# Autodesk Inventor assembly: structure_channel
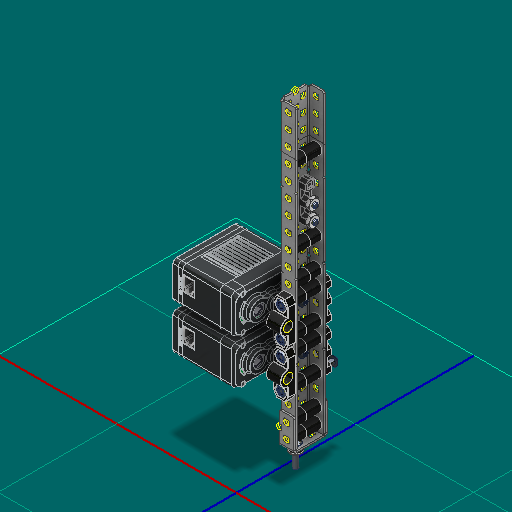
[picture p0: Inventor's stored thumbnail of the model, 512x512]
Saved by Autodesk Inventor 2025 (Build 290162000, 162)
## iProperties
Created: 2024-08-18
Part Number: structure_channel
Document SubType Name: Assembly
Designer: averey
Author: averey
## Documents named in this file (21)
- C:\Users\avere\vex_robotics_high_stakes\hardware\cad\ATLAS\tower\structure\structure_channel.iam
- C:\Users\avere\vex_robotics_high_stakes\hardware\cad\VEX-CAD-Inventor\Structure\C Channel\Aluminum 1x2x1\Alu C 1x2x1x20.ipt
- C:\Users\avere\vex_robotics_high_stakes\hardware\cad\VEX-CAD-Inventor\Structure\C Channel\Aluminum 2x2x2\Alu C 2x2x2x1.ipt
- C:\Users\avere\vex_robotics_high_stakes\hardware\cad\VEX-CAD-Inventor\Motion\Spacers\Spacer Nylon .375 OD\NSpacer .375 OD x .375.ipt
- C:\Users\avere\vex_robotics_high_stakes\hardware\cad\VEX-CAD-Inventor\Motion\Spacers\Spacer Nylon .375 OD.ipt
- C:\Users\avere\vex_robotics_high_stakes\hardware\cad\VEX-CAD-Inventor\Motion\Spacers\Spacer Nylon .375 OD\NSpacer .375 OD x .500.ipt
- C:\Users\avere\vex_robotics_high_stakes\hardware\cad\VEX-CAD-Inventor\Structure\C Channel\Aluminum 1x2x1\Alu C 1x2x1x17.ipt
- C:\Users\avere\vex_robotics_high_stakes\hardware\cad\VEX-CAD-Inventor\Motion\Spacers\Spacer Nylon .375 OD\NSpacer .375 OD x .125.ipt
- C:\Users\avere\vex_robotics_high_stakes\hardware\cad\VEX-CAD-Inventor\Motion\Spacers\Washer Steel\SWasher .375 OD x .015625.ipt
- C:\Users\avere\vex_robotics_high_stakes\hardware\cad\VEX-CAD-Inventor\Motion\Spacers\Washer Steel.ipt
- C:\Users\avere\vex_robotics_high_stakes\hardware\cad\VEX-CAD-Inventor\Motion\Spacers\Washer Steel\SWasher .375 OD x .031250.ipt
- C:\Users\avere\vex_robotics_high_stakes\hardware\cad\VEX-CAD-Inventor\Structure\Hardware\Screw Steel - Star\SScrew Star Smooth .750.ipt
- C:\Users\avere\vex_robotics_high_stakes\hardware\cad\VEX-CAD-Inventor\Structure\Hardware\Screw Steel - Star.ipt
- C:\Users\avere\vex_robotics_high_stakes\hardware\cad\VEX-CAD-Inventor\Electronics\Motors with Screws\SteelM-StarS.iam
- C:\Users\avere\vex_robotics_high_stakes\hardware\cad\VEX-CAD-Inventor\Electronics\Motors with Screws.iam
- C:\Users\avere\vex_robotics_high_stakes\hardware\cad\VEX-CAD-Inventor\Motion\Shaft HS\HS Pillow Bearing Block.ipt
- C:\Users\avere\vex_robotics_high_stakes\hardware\cad\VEX-CAD-Inventor\Motion\Shaft LS\Bearing Flat.ipt
- C:\Users\avere\vex_robotics_high_stakes\hardware\cad\VEX-CAD-Inventor\Structure\Hardware\Screw Steel - Star\SScrew Star Smooth 1.500.ipt
- C:\Users\avere\vex_robotics_high_stakes\hardware\cad\VEX-CAD-Inventor\Structure\Hardware\Nut Thin Nylock.ipt
- C:\Users\avere\vex_robotics_high_stakes\hardware\cad\_quick_assemblies\bearing_flat_w_hardware_offset.iam
- C:\Users\avere\vex_robotics_high_stakes\hardware\cad\VEX-CAD-Inventor\Structure\Hardware\Screw Steel - Star\SScrew Star Smooth 1.750.ipt
## Components (40 placed, 16 different names)
1. Alu C 1x2x1x20:1 — Angle:1, Angle:2, Mate:5, Insert:1, Mate:6, Insert:3, Insert:5, Insert:6, Mate:7
2. Alu C 2x2x2x1:1 — Insert:1, Mate:6, Insert:9, Insert:10
3. NSpacer .375 OD x .375:1 — Insert:2
4. NSpacer .375 OD x .500:2 — Insert:2, Insert:3
5. NSpacer .375 OD x .375:3 — Insert:4
6. NSpacer .375 OD x .500:4 — Insert:4, Insert:5
7. Alu C 1x2x1x17:1 — Insert:6, Mate:7, Insert:11, Mate:8, Insert:12, Mate:9, Insert:15, Mate:12, Insert:16, Mate:13, Insert:18, Insert:20, Insert:22, Insert:24, Insert:25, Mate:14, Insert:26, Mate:15, Insert:35, Mate:16, Insert:37, Insert:39, Insert:41
8. NSpacer .375 OD x .125:5 — Insert:9
9. SWasher .375 OD x .015625:1
10. SWasher .375 OD x .031250:2
11. SScrew Star Smooth .750:1 — Insert:10
12. SteelM-StarS:1 [sub-assembly] — Insert:11, Mate:8
13. SteelM-StarS:2 [sub-assembly] — Insert:12, Mate:9
14. HS Pillow Bearing Block:1 — Insert:15, Mate:12, Insert:31, Insert:32
15. HS Pillow Bearing Block:2 — Insert:16, Mate:13, Insert:33, Insert:34
16. NSpacer .375 OD x .375:6 — Insert:17
17. NSpacer .375 OD x .500:7 — Insert:17, Insert:18
18. NSpacer .375 OD x .375:8
19. NSpacer .375 OD x .500:9 — Insert:20
20. NSpacer .375 OD x .375:10
21. NSpacer .375 OD x .500:11 — Insert:22
22. NSpacer .375 OD x .375:12
23. NSpacer .375 OD x .500:13 — Insert:24
24. Bearing Flat:1 — Insert:25, Mate:14, Insert:29, Insert:42
25. Bearing Flat:2 — Insert:26, Mate:15, Insert:27, Insert:28
26. SScrew Star Smooth 1.500:2 — Insert:27
27. SScrew Star Smooth 1.500:3 — Insert:28
28. SScrew Star Smooth 1.500:5 — Insert:29
29. Nut Thin Nylock:1 — Insert:34
30. Nut Thin Nylock:2 — Insert:32
31. Nut Thin Nylock:3 — Insert:33
32. Nut Thin Nylock:4 — Insert:31
33. bearing_flat_w_hardware_offset:1 [sub-assembly] — Insert:35, Mate:16
34. NSpacer .375 OD x .375:14 — Insert:38
35. NSpacer .375 OD x .500:15 — Insert:38, Insert:39
36. NSpacer .375 OD x .375:16 — Insert:36
37. NSpacer .375 OD x .500:17 — Insert:36, Insert:37
38. NSpacer .375 OD x .375:18
39. NSpacer .375 OD x .500:19 — Insert:41
40. SScrew Star Smooth 1.750:6 — Insert:42
## Relationships (51: Insert 39, Mate 10, Angle 2)
- Angle:1 (0 deg): Alu C 1x2x1x20:1
- Angle:2 (0 deg): Alu C 1x2x1x20:1
- Mate:5 (49.6316 mm): Alu C 1x2x1x20:1
- Insert:1: Alu C 1x2x1x20:1 ↔ Alu C 2x2x2x1:1
- Mate:6: Alu C 1x2x1x20:1 ↔ Alu C 2x2x2x1:1
- Insert:2: NSpacer .375 OD x .375:1 ↔ NSpacer .375 OD x .500:2
- Insert:3: Alu C 1x2x1x20:1 ↔ NSpacer .375 OD x .500:2
- Insert:4: NSpacer .375 OD x .375:3 ↔ NSpacer .375 OD x .500:4
- Insert:5: Alu C 1x2x1x20:1 ↔ NSpacer .375 OD x .500:4
- Insert:6: Alu C 1x2x1x20:1 ↔ Alu C 1x2x1x17:1
- Mate:7: Alu C 1x2x1x20:1 ↔ Alu C 1x2x1x17:1
- [Insert]: SWasher .375 OD x .015625:1 ↔ SWasher .375 OD x .031250:2
- [Insert]: NSpacer .375 OD x .125:5 ↔ SWasher .375 OD x .031250:2
- Insert:9: Alu C 2x2x2x1:1 ↔ NSpacer .375 OD x .125:5
- Insert:10: Alu C 2x2x2x1:1 ↔ SScrew Star Smooth .750:1
- Insert:11: Alu C 1x2x1x17:1 ↔ SteelM-StarS:1
- Mate:8: Alu C 1x2x1x17:1 ↔ SteelM-StarS:1
- Insert:12: Alu C 1x2x1x17:1 ↔ SteelM-StarS:2
- Mate:9: Alu C 1x2x1x17:1 ↔ SteelM-StarS:2
- Insert:15: Alu C 1x2x1x17:1 ↔ HS Pillow Bearing Block:1
- Mate:12: Alu C 1x2x1x17:1 ↔ HS Pillow Bearing Block:1
- Insert:16: Alu C 1x2x1x17:1 ↔ HS Pillow Bearing Block:2
- Mate:13: Alu C 1x2x1x17:1 ↔ HS Pillow Bearing Block:2
- Insert:17: NSpacer .375 OD x .375:6 ↔ NSpacer .375 OD x .500:7
- Insert:18: Alu C 1x2x1x17:1 ↔ NSpacer .375 OD x .500:7
- [Insert]: NSpacer .375 OD x .375:8 ↔ NSpacer .375 OD x .500:9
- Insert:20: Alu C 1x2x1x17:1 ↔ NSpacer .375 OD x .500:9
- [Insert]: NSpacer .375 OD x .375:10 ↔ NSpacer .375 OD x .500:11
- Insert:22: Alu C 1x2x1x17:1 ↔ NSpacer .375 OD x .500:11
- [Insert]: NSpacer .375 OD x .375:12 ↔ NSpacer .375 OD x .500:13
- Insert:24: Alu C 1x2x1x17:1 ↔ NSpacer .375 OD x .500:13
- Insert:25: Alu C 1x2x1x17:1 ↔ Bearing Flat:1
- Mate:14: Alu C 1x2x1x17:1 ↔ Bearing Flat:1
- Insert:26: Alu C 1x2x1x17:1 ↔ Bearing Flat:2
- Mate:15: Alu C 1x2x1x17:1 ↔ Bearing Flat:2
- Insert:27: Bearing Flat:2 ↔ SScrew Star Smooth 1.500:2
- Insert:28: Bearing Flat:2 ↔ SScrew Star Smooth 1.500:3
- Insert:29: Bearing Flat:1 ↔ SScrew Star Smooth 1.500:5
- Insert:31: HS Pillow Bearing Block:1 ↔ Nut Thin Nylock:4
- Insert:32: HS Pillow Bearing Block:1 ↔ Nut Thin Nylock:2
- Insert:33: HS Pillow Bearing Block:2 ↔ Nut Thin Nylock:3
- Insert:34: HS Pillow Bearing Block:2 ↔ Nut Thin Nylock:1
- Insert:35: Alu C 1x2x1x17:1 ↔ bearing_flat_w_hardware_offset:1
- Mate:16: Alu C 1x2x1x17:1 ↔ bearing_flat_w_hardware_offset:1
- Insert:36: NSpacer .375 OD x .375:16 ↔ NSpacer .375 OD x .500:17
- Insert:37: Alu C 1x2x1x17:1 ↔ NSpacer .375 OD x .500:17
- Insert:38: NSpacer .375 OD x .375:14 ↔ NSpacer .375 OD x .500:15
- Insert:39: Alu C 1x2x1x17:1 ↔ NSpacer .375 OD x .500:15
- [Insert]: NSpacer .375 OD x .375:18 ↔ NSpacer .375 OD x .500:19
- Insert:41: Alu C 1x2x1x17:1 ↔ NSpacer .375 OD x .500:19
- Insert:42 (6.35 mm): Bearing Flat:1 ↔ SScrew Star Smooth 1.750:6
## Named parameters: d5_d2 = 0 mm, d6_d3 = 0 mm, d43_d41 = 0 mm, d45_d43_d41 = 0 mm, d47_d43_d41 = 0 mm, d67_d65 = 0 mm
